(part 1 of 3)
# Autodesk Inventor assembly: printer
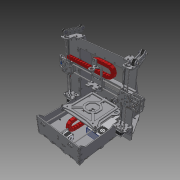
[picture p0: Inventor's stored thumbnail of the model, 180x180]
Saved by Autodesk Inventor 2014 (Build 180170000, 170)
## iProperties
Created: 2013-12-06
Part Number: printer
Document SubType Name: Assembly
Designer: buben
Author: buben
## Documents named in this file (52)
- C:\Users\buben\Documents\GitHub\bacon\inventor files\assemblies\printer.iam
- C:\Users\buben\Documents\GitHub\bacon\inventor files\printer parts\brace_left.ipt
- C:\Users\buben\Documents\GitHub\bacon\inventor files\printer parts\frame.ipt
- C:\Users\buben\Documents\GitHub\bacon\inventor files\printer parts\z_motor_mount.ipt
- C:\Users\buben\Documents\GitHub\bacon\inventor files\printer parts\z_rod_stopper_bottom.ipt
- C:\Users\buben\Documents\GitHub\bacon\inventor files\utils\washer_m4.ipt
- C:\Users\buben\Documents\Inventor\Content Center Files\R2014\en-US\ISO 4762(2)\ISO 4762 - M4 x 20ISO.ipt
- C:\Users\buben\Documents\Inventor\Content Center Files\R2014\en-US\ISO 7040\ISO 7040 - M4.ipt
- C:\Users\buben\Documents\GitHub\bacon\inventor files\3rd party components\nema_17_stepper\Imported Components\NEMA 17\NEMA 17.iam
- C:\Users\buben\Documents\GitHub\bacon\inventor files\utils\washer_m3.ipt
- C:\Users\buben\Documents\Inventor\Content Center Files\R2014\en-US\ISO 4762(2)\ISO 4762 - M3 x 20ISO.ipt
- C:\Users\buben\Documents\GitHub\bacon\inventor files\utils\z_axis_rod.ipt
- C:\Users\buben\Documents\GitHub\bacon\inventor files\printer parts\z_motor_brace.ipt
- C:\Users\buben\Documents\GitHub\bacon\inventor files\utils\z_threaded_rod.ipt
- C:\Users\buben\Documents\GitHub\bacon\inventor files\printer parts\frame_brace_top.ipt
- C:\Users\buben\Documents\GitHub\bacon\inventor files\printer parts\front.ipt
- C:\Users\buben\Documents\GitHub\bacon\inventor files\printer parts\z_axis_top.ipt
- C:\Users\buben\Documents\GitHub\bacon\inventor files\printer parts\bottom.ipt
- C:\Users\buben\Documents\GitHub\bacon\inventor files\printer parts\wiring_brace.ipt
- C:\Users\buben\Documents\GitHub\bacon\inventor files\printer parts\brace_right.ipt
- C:\Users\buben\Documents\GitHub\bacon\inventor files\printer parts\back.ipt
- C:\Users\buben\Documents\GitHub\bacon\inventor files\utils\y_axis_rod.ipt
- C:\Users\buben\Documents\GitHub\bacon\inventor files\utils\z_axis_cable_mount_a.ipt
- C:\Users\buben\Documents\GitHub\bacon\inventor files\assemblies\x_axis.iam
- C:\Users\buben\Documents\GitHub\bacon\inventor files\utils\cable_chain_22.ipt
- C:\Users\buben\Documents\GitHub\bacon\inventor files\utils\z_axis_cable_mount_b.ipt
- C:\Users\buben\Documents\GitHub\bacon\inventor files\assemblies\y_carriage.iam
- C:\Users\buben\Documents\GitHub\bacon\inventor files\utils\y_axis_cable_mount_b.ipt
- C:\Users\buben\Documents\GitHub\bacon\inventor files\utils\x_axis_cable_mount_a.ipt
- C:\Users\buben\Documents\GitHub\bacon\inventor files\3rd party components\switching_power_supply\Imported Components\MW_switching_25A\MW_switching_25A.iam
- C:\Users\buben\Documents\GitHub\bacon\inventor files\3rd party components\bearing_608\Imported Components\608RS\608RS.ipt
- C:\Users\buben\Documents\GitHub\bacon\inventor files\utils\belt_guide.ipt
- C:\Users\buben\Documents\GitHub\bacon\inventor files\utils\washer_m8.ipt
- C:\Users\buben\Documents\GitHub\bacon\inventor files\printer parts\y_carriage_belt_iddler.ipt
- C:\Users\buben\Documents\GitHub\bacon\inventor files\printer parts\y_carriage_belt_iddler_holder.ipt
- C:\Users\buben\Documents\Inventor\Content Center Files\R2014\en-US\ISO 7040\ISO 7040 - M8.ipt
- C:\Users\buben\Documents\Inventor\Content Center Files\R2014\en-US\ISO 4762(2)\ISO 4762 - M8 x 40ISO.ipt
- C:\Users\buben\Documents\Inventor\Content Center Files\R2014\en-US\ISO 4762(2)\ISO 4762 - M4 x 30ISO.ipt
- C:\Users\buben\Documents\GitHub\bacon\inventor files\printer parts\y_motor_mount.ipt
- C:\Users\buben\Documents\GitHub\bacon\inventor files\printer parts\y_motor_mount_brace.ipt
- C:\Users\buben\Documents\GitHub\bacon\inventor files\printer parts\motor_spacer.ipt
- C:\Users\buben\Documents\GitHub\bacon\inventor files\3rd party components\nema_17_stepper\Imported Components\NEMA 17 with T5 Pulley\NEMA 17 with T5 Pulley.iam
- C:\Users\buben\Documents\GitHub\bacon\inventor files\printer parts\rope_mount_a.ipt
- C:\Users\buben\Documents\GitHub\bacon\inventor files\printer parts\rope_mount_b.ipt
- C:\Users\buben\Documents\GitHub\bacon\inventor files\printer parts\z_axis_top_brace.ipt
- C:\Users\buben\Documents\GitHub\bacon\inventor files\printer parts\rope_mount_holder.ipt
- C:\Users\buben\Documents\GitHub\bacon\inventor files\utils\rope_pulley.ipt
- C:\Users\buben\Documents\Inventor\Content Center Files\R2014\en-US\ISO 4762(2)\ISO 4762 - M4 x 35ISO.ipt
- C:\Users\buben\Documents\GitHub\bacon\inventor files\printer parts\z_axis_top_cap.ipt
- C:\Users\buben\Documents\GitHub\bacon\inventor files\printer parts\y_axis_cap.ipt
- C:\Users\buben\Documents\GitHub\bacon\inventor files\3rd party components\iec_plug_socket\Imported Components\IEC inlet\IEC inlet.ipt
- C:\Users\buben\Documents\Inventor\Content Center Files\R2014\en-US\ANSI B18.6.5M(01)\ANSI B18.6.5M - 2.9x1 x 8(4).ipt
## Components (526 placed, 51 different names)
1. brace_left:1 — Mate:1, Mate:2, Flush:1, Mate:3, Mate:4, Mate:5, Mate:71, Mate:73, Flush:6, Flush:7, Mate:80, Flush:8, Mate:85, Mate:111, Mate:113, Mate:115, Mate:177, Mate:179, Mate:181, Mate:241, Mate:243, Mate:245, Mate:247, Mate:249, Mate:276, Mate:277, Mate:278, Mate:279, Mate:280, Mate:281, Mate:282, Mate:283, Mate:284, Mate:285, Mate:367, Mate:395, Mate:396, Mate:398, Mate:400, Mate:427, Mate:665
2. frame:1 — Mate:3, Mate:4, Mate:5, Mate:6, Flush:2, Flush:3, Mate:7, Flush:4, Flush:5, Mate:70, Mate:72, Mate:74, Mate:75, Mate:76, Mate:77, Mate:78, Mate:79, Mate:84, Flush:9, Mate:86, Flush:10, Mate:87, Mate:88, Mate:211, Mate:212, Mate:213, Mate:214, Mate:215, Mate:216, Mate:217, Mate:218, Mate:219, Mate:220, Mate:221, Mate:222, Mate:223, Mate:224, Mate:225, Mate:226, Mate:227, Mate:228, Mate:229, Mate:230, Mate:333, Mate:334, Mate:335, Mate:336, Mate:337, Mate:338, Mate:343, Mate:344, Mate:345, Mate:346, Mate:347, Mate:348, Mate:391, Mate:397, Mate:401, Mate:402, Mate:428, Mate:639, Mate:640, Mate:642, Mate:644, Mate:661, Mate:662, Mate:663, Mate:664, Mate:669, Mate:671, Mate:677, Mate:683
3. z_motor_mount:1 — Mate:6, Flush:2, Flush:3, Mate:8, Mate:9, Mate:10, Mate:14, Mate:15, Mate:16, Mate:17, Mate:44, Mate:45, Mate:46, Mate:47, Mate:52, Mate:53, Mate:54, Mate:55, Insert:13, Mate:63, Mate:64, Mate:65, Mate:339, Mate:340, Mate:341, Mate:342, Mate:359, Mate:361
4. z_motor_mount:2 — Mate:7, Flush:4, Flush:5, Mate:11, Mate:12, Mate:13, Mate:22, Mate:23, Mate:24, Mate:25, Mate:48, Mate:49, Mate:50, Mate:51, Mate:56, Mate:57, Mate:58, Mate:59, Insert:14, Mate:60, Mate:61, Mate:62, Mate:331, Mate:332, Mate:349, Mate:350, Mate:355, Mate:357
5. z_rod_stopper_bottom:1 — Mate:8, Mate:9, Mate:10, Mate:18, Mate:20, Mate:38, Mate:39, Mate:40
6. z_rod_stopper_bottom:2 — Mate:11, Mate:12, Mate:13, Mate:26, Mate:28, Mate:41, Mate:42, Mate:43
7. CSN 02 1702 B B 4,3:1 — Mate:22, Mate:23, Insert:4
8. CSN 02 1702 B B 4,3:2 — Mate:26, Mate:27, Mate:34
9. CSN 02 1702 B B 4,3:3 — Mate:18, Mate:19, Mate:30
10. CSN 02 1702 B B 4,3:4 — Mate:20, Mate:21, Mate:32
11. CSN 02 1702 B B 4,3:5 — Mate:14, Mate:16, Insert:1
12. CSN 02 1702 B B 4,3:6 — Mate:15, Mate:17, Insert:2
13. CSN 02 1702 B B 4,3:7 — Mate:28, Mate:29, Mate:36
14. CSN 02 1702 B B 4,3:8 — Mate:24, Mate:25, Insert:3
15. ISO 4762 M4 x 20:1 — Insert:4, Mate:29, Mate:37
16. ISO 4762 M4 x 20:2 — Insert:3, Mate:27, Mate:35
17. ISO 4762 M4 x 20:3 — Insert:2, Mate:19, Mate:31
18. ISO 4762 M4 x 20:4 — Insert:1, Mate:21, Mate:33
19. DIN EN ISO 7040 M4:1 — Mate:36, Mate:37
20. DIN EN ISO 7040 M4:2 — Mate:34, Mate:35
21. DIN EN ISO 7040 M4:3 — Mate:32, Mate:33
22. DIN EN ISO 7040 M4:4 — Mate:30, Mate:31
23. NEMA 17:1 [sub-assembly] — Mate:38, Mate:39, Mate:40, Mate:66, Mate:67
24. NEMA 17:2 [sub-assembly] — Mate:41, Mate:42, Mate:43, Mate:68, Mate:69
25. CSN 02 1702 B B 3,2:1 — Mate:45, Mate:53, Insert:8
26. CSN 02 1702 B B 3,2:2 — Mate:48, Mate:57, Insert:10
27. CSN 02 1702 B B 3,2:3 — Mate:49, Mate:59, Insert:11
28. CSN 02 1702 B B 3,2:4 — Mate:50, Mate:58, Insert:12
29. CSN 02 1702 B B 3,2:5 — Mate:51, Mate:56, Insert:9
30. CSN 02 1702 B B 3,2:6 — Mate:46, Mate:55, Insert:7
31. CSN 02 1702 B B 3,2:7 — Mate:47, Mate:54, Insert:5
32. CSN 02 1702 B B 3,2:8 — Mate:44, Mate:52, Insert:6
33. ISO 4762 M3 x 20:1 — Insert:12
34. ISO 4762 M3 x 20:2 — Insert:11
35. ISO 4762 M3 x 20:3 — Insert:10
36. ISO 4762 M3 x 20:4 — Insert:9
37. ISO 4762 M3 x 20:5 — Insert:8
38. ISO 4762 M3 x 20:6 — Insert:7
39. ISO 4762 M3 x 20:7 — Insert:6
40. ISO 4762 M3 x 20:8 — Insert:5
41. z_axis_rod:1 — Insert:14, Mate:434
42. z_axis_rod:2 — Insert:13, Mate:433
43. z_motor_brace:1 — Mate:60, Mate:61, Mate:62, Mate:351, Mate:369
44. z_motor_brace:2 — Mate:63, Mate:64, Mate:65, Mate:363, Mate:365
45. z_threaded_rod:1 — Mate:66, Mate:67
46. z_threaded_rod:2 — Mate:68, Mate:69
47. frame_brace_top:1 — Mate:70, Mate:71, Mate:72, Mate:403, Mate:405, Mate:429
48. front:1 — Mate:73, Flush:6, Flush:7, Mate:81, Insert:15, Insert:16, Mate:91, Mate:92, Mate:93, Mate:94, Mate:95, Mate:96, Mate:97, Mate:98, Mate:99, Mate:100, Mate:101, Mate:102, Mate:103, Mate:104, Mate:105, Mate:106, Mate:107, Mate:108, Mate:109, Mate:110, Mate:495, Mate:496, Mate:497, Mate:498, Mate:499, Mate:500, Mate:501, Mate:735, Mate:736, Mate:743, Mate:744, Mate:745, Mate:746, Mate:767, Mate:768, Mate:769, Mate:770
49. z_axis_top:1 — Mate:74, Mate:75, Mate:76, Mate:527, Flush:15, Mate:528, Mate:529, Flush:16, Flush:17, Mate:641, Mate:645, Mate:646, Mate:647, Mate:648, Mate:705, Mate:706, Mate:707, Mate:719, Mate:721
50. z_axis_top:2 — Mate:77, Mate:78, Mate:79, Mate:539, Mate:540, Mate:541, Mate:542, Mate:543, Mate:544, Mate:643, Mate:649, Mate:650, Mate:651, Mate:652, Mate:708, Mate:709, Mate:710, Mate:723, Mate:725
51. bottom:1 — Mate:80, Mate:81, Flush:8, Mate:89, Flush:11, Flush:13, Mate:117, Mate:119, Mate:121, Mate:123, Mate:183, Mate:185, Mate:187, Mate:189, Mate:291, Mate:293, Mate:295, Mate:297, Mate:299, Mate:301, Mate:303, Mate:305, Mate:307, Mate:309, Mate:443, Mate:444, Mate:445
52. wiring_brace:1 — Mate:84, Flush:9, Mate:85, Mate:409, Mate:413
53. wiring_brace:2 — Mate:86, Flush:10, Mate:87, Mate:407, Mate:411
54. brace_right:1 — Mate:88, Mate:89, Flush:11, Mate:90, Flush:12, Mate:125, Mate:127, Mate:129, Mate:171, Mate:173, Mate:175, Mate:231, Mate:233, Mate:235, Mate:237, Mate:239, Mate:271, Mate:272, Mate:273, Mate:274, Mate:275, Mate:286, Mate:287, Mate:288, Mate:289, Mate:290, Mate:353, Mate:392, Mate:393, Mate:394, Mate:399, Mate:446, Mate:675, Mate:795, Mate:796, Mate:797
55. back:1 — Mate:90, Flush:12, Flush:13, Mate:151, Mate:152, Mate:153, Mate:154, Mate:155, Mate:156, Mate:157, Mate:158, Mate:159, Mate:160, Mate:161, Mate:162, Mate:163, Mate:164, Mate:165, Mate:166, Mate:167, Mate:168, Mate:169, Mate:170, Mate:442, Mate:447, Mate:469, Mate:477, Mate:478, Mate:479, Mate:480, Mate:481, Mate:482, Mate:737, Mate:738, Mate:739, Mate:740, Mate:741, Mate:742, Mate:759, Mate:760, Mate:761, Mate:762
56. y_axis_rod:1 — Insert:16, Mate:441
57. y_axis_rod:2 — Insert:15, Mate:440
58. CSN 02 1702 B B 4,3:9 — Mate:97, Mate:107, Insert:23
59. CSN 02 1702 B B 4,3:10 — Mate:98, Mate:108, Insert:24
60. CSN 02 1702 B B 4,3:11 — Mate:99, Mate:109, Insert:25
61. CSN 02 1702 B B 4,3:12 — Mate:129, Mate:130, Mate:149
62. CSN 02 1702 B B 4,3:13 — Mate:94, Mate:104, Insert:20
63. CSN 02 1702 B B 4,3:14 — Mate:95, Mate:105, Insert:21
64. CSN 02 1702 B B 4,3:15 — Mate:96, Mate:106, Insert:22
65. CSN 02 1702 B B 4,3:16 — Mate:93, Mate:103, Insert:19
66. CSN 02 1702 B B 4,3:17 — Mate:92, Mate:102, Insert:18
67. CSN 02 1702 B B 4,3:18 — Mate:91, Mate:101, Insert:17
68. CSN 02 1702 B B 4,3:19 — Mate:127, Mate:128, Mate:147
69. CSN 02 1702 B B 4,3:20 — Mate:117, Mate:118, Mate:137
70. CSN 02 1702 B B 4,3:21 — Mate:115, Mate:116, Mate:135
71. CSN 02 1702 B B 4,3:22 — Mate:100, Mate:110, Insert:26
72. CSN 02 1702 B B 4,3:23 — Mate:125, Mate:126, Mate:145
73. CSN 02 1702 B B 4,3:24 — Mate:121, Mate:122, Mate:141
74. CSN 02 1702 B B 4,3:25 — Mate:113, Mate:114, Mate:133
75. CSN 02 1702 B B 4,3:26 — Mate:123, Mate:124, Mate:143
76. CSN 02 1702 B B 4,3:27 — Mate:119, Mate:120, Mate:139
77. CSN 02 1702 B B 4,3:28 — Mate:111, Mate:112, Mate:131
78. ISO 4762 M4 x 20:5 — Insert:17, Mate:112, Mate:132
79. ISO 4762 M4 x 20:6 — Insert:18, Mate:114, Mate:134
80. ISO 4762 M4 x 20:7 — Insert:19, Mate:116, Mate:136
81. ISO 4762 M4 x 20:8 — Insert:20, Mate:118, Mate:138
82. ISO 4762 M4 x 20:9 — Insert:21, Mate:120, Mate:140
83. ISO 4762 M4 x 20:10 — Insert:22, Mate:122, Mate:142
84. ISO 4762 M4 x 20:11 — Insert:23, Mate:124, Mate:144
85. ISO 4762 M4 x 20:12 — Insert:24, Mate:130, Mate:150
86. ISO 4762 M4 x 20:13 — Insert:25, Mate:128, Mate:148
87. ISO 4762 M4 x 20:14 — Insert:26, Mate:126, Mate:146
88. DIN EN ISO 7040 M4:5 — Mate:131, Mate:132
89. DIN EN ISO 7040 M4:6 — Mate:141, Mate:142
90. DIN EN ISO 7040 M4:7 — Mate:143, Mate:144
91. DIN EN ISO 7040 M4:8 — Mate:147, Mate:148
92. DIN EN ISO 7040 M4:9 — Mate:135, Mate:136
93. DIN EN ISO 7040 M4:10 — Mate:145, Mate:146
94. DIN EN ISO 7040 M4:11 — Mate:149, Mate:150
95. DIN EN ISO 7040 M4:12 — Mate:133, Mate:134
96. DIN EN ISO 7040 M4:13 — Mate:137, Mate:138
97. DIN EN ISO 7040 M4:14 — Mate:139, Mate:140
98. CSN 02 1702 B B 4,3:29 — Mate:151, Mate:168, Insert:29
99. CSN 02 1702 B B 4,3:30 — Mate:152, Mate:169, Insert:28
100. CSN 02 1702 B B 4,3:31 — Mate:160, Mate:161, Insert:36
101. CSN 02 1702 B B 4,3:32 — Mate:153, Mate:170, Insert:27
102. CSN 02 1702 B B 4,3:33 — Mate:154, Mate:167, Insert:30
103. CSN 02 1702 B B 4,3:34 — Mate:159, Mate:162, Insert:35
104. CSN 02 1702 B B 4,3:35 — Mate:155, Mate:166, Insert:31
105. CSN 02 1702 B B 4,3:36 — Mate:156, Mate:165, Insert:32
106. CSN 02 1702 B B 4,3:37 — Mate:157, Mate:164, Insert:33
107. CSN 02 1702 B B 4,3:38 — Mate:158, Mate:163, Insert:34
108. CSN 02 1702 B B 4,3:39 — Mate:171, Mate:172, Mate:205
109. CSN 02 1702 B B 4,3:40 — Mate:175, Mate:176, Mate:209
110. CSN 02 1702 B B 4,3:41 — Mate:173, Mate:174, Mate:207
111. CSN 02 1702 B B 4,3:42 — Mate:177, Mate:178, Mate:191
112. CSN 02 1702 B B 4,3:43 — Mate:181, Mate:182, Mate:195
113. CSN 02 1702 B B 4,3:44 — Mate:187, Mate:188, Mate:201
114. CSN 02 1702 B B 4,3:45 — Mate:179, Mate:180, Mate:193
115. CSN 02 1702 B B 4,3:46 — Mate:183, Mate:184, Mate:197
116. CSN 02 1702 B B 4,3:47 — Mate:185, Mate:186, Mate:199
117. CSN 02 1702 B B 4,3:48 — Mate:189, Mate:190, Mate:203
118. ISO 4762 M4 x 20:15 — Insert:27, Mate:178, Mate:192
119. ISO 4762 M4 x 20:16 — Insert:28, Mate:180, Mate:194
120. ISO 4762 M4 x 20:17 — Insert:29, Mate:182, Mate:196
121. ISO 4762 M4 x 20:18 — Insert:30, Mate:184, Mate:198
122. ISO 4762 M4 x 20:19 — Insert:31, Mate:186, Mate:200
123. ISO 4762 M4 x 20:20 — Insert:32, Mate:188, Mate:202
124. ISO 4762 M4 x 20:21 — Insert:33, Mate:190, Mate:204
125. ISO 4762 M4 x 20:22 — Insert:34, Mate:176, Mate:210
126. ISO 4762 M4 x 20:23 — Insert:35, Mate:174, Mate:208
127. ISO 4762 M4 x 20:24 — Insert:36, Mate:172, Mate:206
128. DIN EN ISO 7040 M4:15 — Mate:193, Mate:194
129. DIN EN ISO 7040 M4:16 — Mate:207, Mate:208
130. DIN EN ISO 7040 M4:17 — Mate:191, Mate:192
131. DIN EN ISO 7040 M4:18 — Mate:201, Mate:202
132. DIN EN ISO 7040 M4:19 — Mate:209, Mate:210
133. DIN EN ISO 7040 M4:20 — Mate:205, Mate:206
134. DIN EN ISO 7040 M4:21 — Mate:203, Mate:204
135. DIN EN ISO 7040 M4:22 — Mate:195, Mate:196
136. DIN EN ISO 7040 M4:23 — Mate:197, Mate:198
137. DIN EN ISO 7040 M4:24 — Mate:199, Mate:200
138. CSN 02 1702 B B 4,3:49 — Mate:211, Mate:226, Insert:37
139. CSN 02 1702 B B 4,3:50 — Mate:213, Mate:228, Insert:39
140. CSN 02 1702 B B 4,3:51 — Mate:214, Mate:229, Insert:40
141. CSN 02 1702 B B 4,3:52 — Mate:215, Mate:230, Insert:41
142. CSN 02 1702 B B 4,3:53 — Mate:216, Mate:221, Insert:42
143. CSN 02 1702 B B 4,3:54 — Mate:217, Mate:222, Insert:43
144. CSN 02 1702 B B 4,3:55 — Mate:218, Mate:223, Insert:44
145. CSN 02 1702 B B 4,3:56 — Mate:219, Mate:224, Insert:45
146. CSN 02 1702 B B 4,3:57 — Mate:220, Mate:225, Insert:46
147. CSN 02 1702 B B 4,3:58 — Mate:247, Mate:248, Mate:267
148. CSN 02 1702 B B 4,3:59 — Mate:212, Mate:227, Insert:38
149. CSN 02 1702 B B 4,3:60 — Mate:231, Mate:232, Mate:251
150. CSN 02 1702 B B 4,3:61 — Mate:233, Mate:234, Mate:253
151. CSN 02 1702 B B 4,3:62 — Mate:235, Mate:236, Mate:255
152. CSN 02 1702 B B 4,3:63 — Mate:237, Mate:238, Mate:257
153. CSN 02 1702 B B 4,3:64 — Mate:239, Mate:240, Mate:259
154. CSN 02 1702 B B 4,3:65 — Mate:241, Mate:242, Mate:261
155. CSN 02 1702 B B 4,3:66 — Mate:243, Mate:244, Mate:263
156. CSN 02 1702 B B 4,3:67 — Mate:245, Mate:246, Mate:265
157. CSN 02 1702 B B 4,3:68 — Mate:249, Mate:250, Mate:269
158. ISO 4762 M4 x 20:25 — Insert:37, Mate:232, Mate:252
159. ISO 4762 M4 x 20:26 — Insert:38, Mate:234, Mate:254
160. ISO 4762 M4 x 20:27 — Insert:39, Mate:236, Mate:256
161. ISO 4762 M4 x 20:28 — Insert:40, Mate:238, Mate:258
162. ISO 4762 M4 x 20:29 — Insert:41, Mate:240, Mate:260
163. ISO 4762 M4 x 20:30 — Insert:42, Mate:242, Mate:262
164. ISO 4762 M4 x 20:31 — Insert:43, Mate:244, Mate:264
165. ISO 4762 M4 x 20:32 — Insert:44, Mate:246, Mate:266
166. ISO 4762 M4 x 20:33 — Insert:45, Mate:248, Mate:268
167. ISO 4762 M4 x 20:34 — Insert:46, Mate:250, Mate:270
168. DIN EN ISO 7040 M4:25 — Mate:251, Mate:252
169. DIN EN ISO 7040 M4:26 — Mate:253, Mate:254
170. DIN EN ISO 7040 M4:27 — Mate:255, Mate:256
171. DIN EN ISO 7040 M4:28 — Mate:261, Mate:262
172. DIN EN ISO 7040 M4:29 — Mate:263, Mate:264
173. DIN EN ISO 7040 M4:30 — Mate:267, Mate:268
174. DIN EN ISO 7040 M4:31 — Mate:269, Mate:270
175. DIN EN ISO 7040 M4:32 — Mate:265, Mate:266
176. DIN EN ISO 7040 M4:33 — Mate:259, Mate:260
177. DIN EN ISO 7040 M4:34 — Mate:257, Mate:258
178. CSN 02 1702 B B 4,3:69 — Mate:271, Mate:290, Insert:51
179. CSN 02 1702 B B 4,3:70 — Mate:272, Mate:289, Insert:50
180. CSN 02 1702 B B 4,3:71 — Mate:273, Mate:288, Insert:49
181. CSN 02 1702 B B 4,3:72 — Mate:274, Mate:287, Insert:48
182. CSN 02 1702 B B 4,3:73 — Mate:275, Mate:286, Insert:47
183. CSN 02 1702 B B 4,3:74 — Mate:276, Mate:281, Insert:56
184. CSN 02 1702 B B 4,3:75 — Mate:277, Mate:282, Insert:55
185. CSN 02 1702 B B 4,3:76 — Mate:278, Mate:283, Insert:54
186. CSN 02 1702 B B 4,3:77 — Mate:279, Mate:284, Insert:53
187. CSN 02 1702 B B 4,3:78 — Mate:280, Mate:285, Insert:52
188. CSN 02 1702 B B 4,3:79 — Mate:303, Mate:304, Mate:317
189. CSN 02 1702 B B 4,3:80 — Mate:305, Mate:306, Mate:315
190. CSN 02 1702 B B 4,3:81 — Mate:307, Mate:308, Mate:313
191. CSN 02 1702 B B 4,3:82 — Mate:309, Mate:310, Mate:311
192. CSN 02 1702 B B 4,3:83 — Mate:301, Mate:302, Mate:319
193. CSN 02 1702 B B 4,3:84 — Mate:299, Mate:300, Mate:329
194. CSN 02 1702 B B 4,3:85 — Mate:297, Mate:298, Mate:325
195. CSN 02 1702 B B 4,3:86 — Mate:295, Mate:296, Mate:327
196. CSN 02 1702 B B 4,3:87 — Mate:293, Mate:294, Mate:323
197. CSN 02 1702 B B 4,3:88 — Mate:291, Mate:292, Mate:321
198. ISO 4762 M4 x 20:35 — Insert:56, Mate:300, Mate:330
199. ISO 4762 M4 x 20:36 — Insert:55, Mate:298, Mate:326
200. ISO 4762 M4 x 20:37 — Insert:54, Mate:296, Mate:328
201. ISO 4762 M4 x 20:38 — Insert:53, Mate:294, Mate:324
202. ISO 4762 M4 x 20:39 — Insert:52, Mate:292, Mate:322
203. ISO 4762 M4 x 20:40 — Insert:51, Mate:302, Mate:320
204. ISO 4762 M4 x 20:41 — Insert:50, Mate:304, Mate:318
205. ISO 4762 M4 x 20:42 — Insert:49, Mate:306, Mate:316
206. ISO 4762 M4 x 20:43 — Insert:48, Mate:308, Mate:314
207. ISO 4762 M4 x 20:44 — Insert:47, Mate:310, Mate:312
208. DIN EN ISO 7040 M4:35 — Mate:329, Mate:330
209. DIN EN ISO 7040 M4:36 — Mate:327, Mate:328
210. DIN EN ISO 7040 M4:37 — Mate:321, Mate:322
211. DIN EN ISO 7040 M4:38 — Mate:317, Mate:318
212. DIN EN ISO 7040 M4:39 — Mate:315, Mate:316
213. DIN EN ISO 7040 M4:40 — Mate:313, Mate:314
214. DIN EN ISO 7040 M4:41 — Mate:311, Mate:312
215. DIN EN ISO 7040 M4:42 — Mate:319, Mate:320
216. DIN EN ISO 7040 M4:43 — Mate:323, Mate:324
217. DIN EN ISO 7040 M4:44 — Mate:325, Mate:326
218. CSN 02 1702 B B 4,3:89 — Mate:340, Mate:341, Insert:65
219. CSN 02 1702 B B 4,3:90 — Mate:339, Mate:342, Insert:66
220. CSN 02 1702 B B 4,3:91 — Mate:338, Mate:345, Insert:64
221. CSN 02 1702 B B 4,3:92 — Mate:337, Mate:344, Insert:63
222. CSN 02 1702 B B 4,3:93 — Mate:336, Mate:343, Insert:62
223. CSN 02 1702 B B 4,3:94 — Mate:335, Mate:348, Insert:61
224. CSN 02 1702 B B 4,3:95 — Mate:334, Mate:347, Insert:59
225. CSN 02 1702 B B 4,3:96 — Mate:333, Mate:346, Insert:60
226. CSN 02 1702 B B 4,3:97 — Mate:332, Mate:349, Insert:57
227. CSN 02 1702 B B 4,3:98 — Mate:331, Mate:350, Insert:58
228. CSN 02 1702 B B 4,3:99 — Mate:367, Mate:368, Mate:385
229. CSN 02 1702 B B 4,3:100 — Mate:369, Mate:370, Mate:375
230. CSN 02 1702 B B 4,3:101 — Mate:365, Mate:366, Mate:383
231. CSN 02 1702 B B 4,3:102 — Mate:363, Mate:364, Mate:381
232. CSN 02 1702 B B 4,3:103 — Mate:361, Mate:362, Mate:389
233. CSN 02 1702 B B 4,3:104 — Mate:359, Mate:360, Mate:387
234. CSN 02 1702 B B 4,3:105 — Mate:357, Mate:358, Mate:373
235. CSN 02 1702 B B 4,3:106 — Mate:355, Mate:356, Mate:371
236. CSN 02 1702 B B 4,3:107 — Mate:353, Mate:354, Mate:379
237. CSN 02 1702 B B 4,3:108 — Mate:351, Mate:352, Mate:377
238. ISO 4762 M4 x 20:45 — Insert:64, Mate:364, Mate:382
239. ISO 4762 M4 x 20:46 — Insert:65, Mate:366, Mate:384
240. ISO 4762 M4 x 20:47 — Insert:66, Mate:368, Mate:386
241. ISO 4762 M4 x 20:48 — Insert:63, Mate:360, Mate:388
242. ISO 4762 M4 x 20:49 — Insert:62, Mate:362, Mate:390
243. ISO 4762 M4 x 20:50 — Insert:61, Mate:370, Mate:376
244. ISO 4762 M4 x 20:51 — Insert:60, Mate:358, Mate:374
245. ISO 4762 M4 x 20:52 — Insert:59, Mate:356, Mate:372
246. ISO 4762 M4 x 20:53 — Insert:58, Mate:354, Mate:380
247. ISO 4762 M4 x 20:54 — Insert:57, Mate:352, Mate:378
248. DIN EN ISO 7040 M4:45 — Mate:389, Mate:390
249. DIN EN ISO 7040 M4:46 — Mate:387, Mate:388
250. DIN EN ISO 7040 M4:47 — Mate:385, Mate:386
251. DIN EN ISO 7040 M4:48 — Mate:383, Mate:384
252. DIN EN ISO 7040 M4:49 — Mate:381, Mate:382
253. DIN EN ISO 7040 M4:50 — Mate:379, Mate:380
254. DIN EN ISO 7040 M4:51 — Mate:377, Mate:378
255. DIN EN ISO 7040 M4:52 — Mate:373, Mate:374
256. DIN EN ISO 7040 M4:53 — Mate:375, Mate:376
257. DIN EN ISO 7040 M4:54 — Mate:371, Mate:372
258. CSN 02 1702 B B 4,3:109 — Mate:393, Mate:394, Insert:67
259. CSN 02 1702 B B 4,3:110 — Mate:397, Mate:402, Insert:69
260. CSN 02 1702 B B 4,3:111 — Mate:398, Mate:400, Insert:71
261. CSN 02 1702 B B 4,3:112 — Mate:407, Mate:408, Mate:415
262. CSN 02 1702 B B 4,3:113 — Mate:403, Mate:404, Mate:425
263. CSN 02 1702 B B 4,3:114 — Mate:395, Mate:396, Insert:72
264. CSN 02 1702 B B 4,3:115 — Mate:392, Mate:399, Insert:70
265. CSN 02 1702 B B 4,3:116 — Mate:405, Mate:406, Mate:419
266. CSN 02 1702 B B 4,3:117 — Mate:411, Mate:412, Mate:417
267. CSN 02 1702 B B 4,3:118 — Mate:413, Mate:414, Mate:421
268. CSN 02 1702 B B 4,3:119 — Mate:409, Mate:410, Mate:423
269. CSN 02 1702 B B 4,3:120 — Mate:391, Mate:401, Insert:68
270. ISO 4762 M4 x 20:55 — Insert:72, Mate:404, Mate:426
271. ISO 4762 M4 x 20:56 — Insert:71, Mate:410, Mate:424
272. ISO 4762 M4 x 20:57 — Insert:70, Mate:408, Mate:416
273. ISO 4762 M4 x 20:58 — Insert:69, Mate:414, Mate:422
274. ISO 4762 M4 x 20:59 — Insert:68, Mate:412, Mate:418
275. ISO 4762 M4 x 20:60 — Insert:67, Mate:406, Mate:420
276. DIN EN ISO 7040 M4:55 — Mate:425, Mate:426
277. DIN EN ISO 7040 M4:56 — Mate:423, Mate:424
278. DIN EN ISO 7040 M4:57 — Mate:421, Mate:422
279. DIN EN ISO 7040 M4:58 — Mate:419, Mate:420
280. DIN EN ISO 7040 M4:59 — Mate:417, Mate:418
281. DIN EN ISO 7040 M4:60 — Mate:415, Mate:416
282. z_axis_cable_mount_a:1 — Mate:427, Mate:428, Mate:429, Insert:96, Angle:24
283. x_axis:1 [sub-assembly] — Mate:433, Mate:434, Mate:435, Flush:14
284. cable_chain_22:1 — Insert:96, Angle:24
285. cable_chain_22:2
286. cable_chain_22:3
287. cable_chain_22:4
288. cable_chain_22:5
289. cable_chain_22:6
290. cable_chain_22:7
291. cable_chain_22:8
292. cable_chain_22:9
293. cable_chain_22:10
294. cable_chain_22:11
295. cable_chain_22:12
296. cable_chain_22:13
297. cable_chain_22:14
298. cable_chain_22:15
299. cable_chain_22:16
300. cable_chain_22:17
301. cable_chain_22:18
302. cable_chain_22:19
303. cable_chain_22:20 — Insert:97, Angle:25
304. z_axis_cable_mount_b:1 — Insert:97, Mate:435, Flush:14, Angle:25
305. y_carriage:1 [sub-assembly] — Mate:436, Mate:437, Mate:438, Mate:440, Mate:441
306. y_axis_cable_mount_b:1 — Mate:436, Mate:437, Mate:438, Insert:121, Angle:65
307. cable_chain_22:22 — Insert:122, Angle:66
308. cable_chain_22:23
309. cable_chain_22:24
310. cable_chain_22:25
311. cable_chain_22:26
312. cable_chain_22:27
313. cable_chain_22:28
314. cable_chain_22:29
315. cable_chain_22:30
316. cable_chain_22:31 — Mate:444
317. cable_chain_22:32
318. cable_chain_22:33
319. cable_chain_22:34
320. cable_chain_22:35
321. cable_chain_22:36
322. cable_chain_22:37
323. cable_chain_22:38
324. cable_chain_22:39
325. cable_chain_22:40
326. cable_chain_22:41
327. cable_chain_22:42
328. cable_chain_22:43
329. cable_chain_22:44 — Insert:121, Angle:65
330. x_axis_cable_mount_a:1 — Insert:122, Angle:66, Mate:442, Mate:443
331. MW_switching_25A:1 [sub-assembly] — Mate:445, Mate:446, Mate:447
332. 608RS:1 — Mate:448, Mate:449, Mate:450, Mate:453, Mate:454, Mate:457, Mate:458
333. belt_guide:1 — Mate:448, Mate:449, Mate:451, Mate:452
334. belt_guide:2 — Mate:450, Mate:451, Mate:452
335. CSN 02 1702 B B 8,4:1 — Mate:453, Mate:454, Mate:455, Mate:456
336. CSN 02 1702 B B 8,4:2 — Mate:455, Mate:456, Mate:461, Mate:462
337. CSN 02 1702 B B 8,4:3 — Mate:457, Mate:458, Mate:459, Mate:460
338. CSN 02 1702 B B 8,4:4 — Mate:459, Mate:460
339. y_carriage_belt_iddler:1 — Mate:461, Mate:462, Mate:463, Mate:464, Mate:465, Mate:472
340. y_carriage_belt_iddler:2 — Mate:466, Mate:467, Mate:468, Mate:469, Mate:470, Mate:471, Mate:477, Mate:478
341. y_carriage_belt_iddler_holder:1 — Mate:463, Mate:464, Mate:465, Mate:466, Mate:467, Mate:468, Mate:483, Mate:484
342. CSN 02 1702 B B 8,4:5 — Mate:470, Mate:471, Insert:123
343. CSN 02 1702 B B 8,4:6 — Mate:472, Mate:474, Mate:475
344. DIN EN ISO 7040 M8:1 — Mate:474, Mate:476
345. ISO 4762 M8 x 40:1 — Insert:123, Mate:475, Mate:476
346. CSN 02 1702 B B 4,3:121 — Mate:483, Mate:485, Mate:487
347. CSN 02 1702 B B 4,3:122 — Mate:484, Mate:486, Mate:489
348. CSN 02 1702 B B 4,3:123 — Mate:480, Mate:481, Insert:125
349. CSN 02 1702 B B 4,3:124 — Mate:479, Mate:482, Insert:124
350. ISO 4762 M4 x 30:1 — Insert:124, Mate:485, Mate:488
351. ISO 4762 M4 x 30:2 — Insert:125, Mate:486, Mate:490
352. DIN EN ISO 7040 M4:61 — Mate:487, Mate:488
353. DIN EN ISO 7040 M4:62 — Mate:489, Mate:490
354. y_motor_mount:1 — Mate:491, Mate:492, Mate:493, Mate:494, Tangent:1, Tangent:2, Mate:495, Mate:496, Mate:502, Mate:503, Mate:508, Mate:519, Mate:520, Mate:521, Mate:522
355. y_motor_mount_brace:1 — Mate:491, Mate:492, Mate:493, Mate:497, Mate:504, Mate:505
356. motor_spacer:1 — Mate:494, Tangent:1, Tangent:2, Mate:516, Mate:517, Mate:518, Mate:523, Mate:524, Mate:525, Mate:526
357. CSN 02 1702 B B 4,3:125 — Mate:504, Mate:507, Mate:512
358. CSN 02 1702 B B 4,3:126 — Mate:508, Mate:509, Mate:514
359. CSN 02 1702 B B 4,3:127 — Mate:498, Mate:501, Insert:127
360. CSN 02 1702 B B 4,3:128 — Mate:499, Mate:500, Insert:126
361. CSN 02 1702 B B 4,3:129 — Mate:505, Mate:506, Mate:510
362. CSN 02 1702 B B 4,3:130 — Mate:502, Mate:503, Insert:128
363. ISO 4762 M4 x 20:61 — Insert:126, Mate:509, Mate:515
364. ISO 4762 M4 x 20:62 — Insert:127, Mate:506, Mate:511
365. ISO 4762 M4 x 20:63 — Insert:128, Mate:507, Mate:513
366. DIN EN ISO 7040 M4:63 — Mate:512, Mate:513
367. DIN EN ISO 7040 M4:64 — Mate:514, Mate:515
368. DIN EN ISO 7040 M4:65 — Mate:510, Mate:511
369. NEMA 17 with T5 Pulley:1 [sub-assembly] — Mate:516, Mate:517, Mate:518
370. CSN 02 1702 B B 3,2:9 — Mate:519, Mate:523, Insert:130
371. CSN 02 1702 B B 3,2:10 — Mate:520, Mate:524, Insert:129
372. CSN 02 1702 B B 3,2:11 — Mate:521, Mate:525, Insert:132
373. CSN 02 1702 B B 3,2:12 — Mate:522, Mate:526, Insert:131
374. ISO 4762 M3 x 20:9 — Insert:132
375. ISO 4762 M3 x 20:10 — Insert:131
376. ISO 4762 M3 x 20:11 — Insert:130
377. ISO 4762 M3 x 20:12 — Insert:129
378. rope_mount_a:1 — Mate:527, Flush:15, Mate:528, Mate:532, Mate:619, Mate:620
379. rope_mount_b:1 — Mate:529, Flush:16, Flush:17, Mate:533, Mate:534, Mate:607, Mate:608, Mate:609, Mate:610, Mate:621, Mate:622, Mate:623, Mate:624
380. rope_mount_holder:1 — Mate:532, Mate:533, Mate:534, Mate:653, Mate:654, Mate:655, Mate:656
381. rope_mount_a:2 — Mate:542, Mate:543, Mate:544, Mate:625, Mate:626
382. rope_mount_b:2 — Mate:539, Mate:540, Mate:541, Mate:545, Mate:546, Mate:547, Mate:611, Mate:612, Mate:613, Mate:614, Mate:615, Mate:616, Mate:617, Mate:618
383. rope_mount_holder:2 — Mate:545, Mate:546, Mate:547, Mate:657, Mate:658, Mate:659, Mate:660
384. 608RS:4 — Mate:550, Mate:556, Mate:559, Mate:564, Mate:565, Mate:566, Mate:567
385. rope_pulley:3 — Mate:557, Mate:558, Mate:559
386. rope_pulley:4 — Mate:550, Mate:556, Mate:557, Mate:558
387. CSN 02 1702 B B 8,4:7 — Mate:560, Mate:561, Mate:564, Mate:565
388. CSN 02 1702 B B 8,4:8 — Mate:560, Mate:561
389. CSN 02 1702 B B 8,4:9 — Mate:562, Mate:563, Mate:566, Mate:567
390. CSN 02 1702 B B 8,4:10 — Mate:562, Mate:563, Mate:613, Mate:614
391. 608RS:5
392. rope_pulley:5
393. rope_pulley:6
394. CSN 02 1702 B B 8,4:11
395. CSN 02 1702 B B 8,4:12
396. CSN 02 1702 B B 8,4:13
397. CSN 02 1702 B B 8,4:14 — Mate:607, Mate:608
398. 608RS:6
399. rope_pulley:7
400. rope_pulley:8
401. CSN 02 1702 B B 8,4:15
402. CSN 02 1702 B B 8,4:16
403. CSN 02 1702 B B 8,4:17
404. CSN 02 1702 B B 8,4:18 — Mate:609, Mate:610
405. 608RS:7
406. rope_pulley:9
407. rope_pulley:10
408. CSN 02 1702 B B 8,4:19
409. CSN 02 1702 B B 8,4:20
410. CSN 02 1702 B B 8,4:21
411. CSN 02 1702 B B 8,4:22 — Mate:611, Mate:612
412. CSN 02 1702 B B 8,4:23 — Mate:626, Mate:628, Mate:631
413. CSN 02 1702 B B 8,4:24 — Mate:625, Mate:627, Mate:633
414. CSN 02 1702 B B 8,4:25 — Mate:623, Mate:624, Insert:136
415. CSN 02 1702 B B 8,4:26 — Mate:621, Mate:622, Insert:135
416. CSN 02 1702 B B 8,4:27 — Mate:620, Mate:630, Mate:635
417. CSN 02 1702 B B 8,4:28 — Mate:619, Mate:629, Mate:637
418. CSN 02 1702 B B 8,4:29 — Mate:617, Mate:618, Insert:134
419. CSN 02 1702 B B 8,4:30 — Mate:615, Mate:616, Insert:133
420. ISO 4762 M8 x 40:2 — Insert:136, Mate:630, Mate:636
421. ISO 4762 M8 x 40:3 — Insert:135, Mate:629, Mate:638
422. ISO 4762 M8 x 40:4 — Insert:134, Mate:628, Mate:632
423. ISO 4762 M8 x 40:5 — Insert:133, Mate:627, Mate:634
424. DIN EN ISO 7040 M8:2 — Mate:637, Mate:638
425. DIN EN ISO 7040 M8:3 — Mate:635, Mate:636
426. DIN EN ISO 7040 M8:4 — Mate:633, Mate:634
427. DIN EN ISO 7040 M8:5 — Mate:631, Mate:632
428. z_axis_top_brace:1 — Mate:642, Mate:643, Mate:644, Mate:673, Mate:681
429. z_axis_top_brace:2 — Mate:639, Mate:640, Mate:641, Mate:667, Mate:679
430. CSN 02 1702 B B 4,3:131 — Mate:651, Mate:652, Insert:139
431. CSN 02 1702 B B 4,3:132 — Mate:659, Mate:660, Insert:146
432. CSN 02 1702 B B 4,3:133 — Mate:657, Mate:658, Insert:145
433. CSN 02 1702 B B 4,3:134 — Mate:655, Mate:656, Insert:143
434. CSN 02 1702 B B 4,3:135 — Mate:645, Mate:646, Insert:137
435. CSN 02 1702 B B 4,3:136 — Mate:649, Mate:650, Insert:140
436. CSN 02 1702 B B 4,3:137 — Mate:647, Mate:648, Insert:138
437. CSN 02 1702 B B 4,3:138 — Mate:653, Mate:654, Insert:144
438. CSN 02 1702 B B 4,3:139 — Mate:661, Mate:662, Insert:141
439. CSN 02 1702 B B 4,3:140 — Mate:671, Mate:672, Mate:701
440. CSN 02 1702 B B 4,3:141 — Mate:675, Mate:676, Mate:703
441. CSN 02 1702 B B 4,3:142 — Mate:665, Mate:666, Mate:685
442. CSN 02 1702 B B 4,3:143 — Mate:673, Mate:674, Mate:697
443. CSN 02 1702 B B 4,3:144 — Mate:669, Mate:670, Mate:687
444. CSN 02 1702 B B 4,3:145 — Mate:667, Mate:668, Mate:691
445. CSN 02 1702 B B 4,3:146 — Mate:663, Mate:664, Insert:142
446. ISO 4762 M4 x 20:64 — Insert:137, Mate:666, Mate:686
447. ISO 4762 M4 x 20:65 — Insert:138, Mate:670, Mate:688
448. ISO 4762 M4 x 20:66 — Insert:139, Mate:672, Mate:702
449. ISO 4762 M4 x 20:67 — Insert:140, Mate:676, Mate:704
450. ISO 4762 M4 x 20:68 — Insert:141, Mate:668, Mate:692
451. ISO 4762 M4 x 20:69 — Insert:142, Mate:674, Mate:698
452. ISO 4762 M4 x 35:1 — Insert:143, Mate:680, Mate:690
453. ISO 4762 M4 x 35:2 — Insert:144, Mate:678, Mate:694
454. ISO 4762 M4 x 35:3 — Insert:145, Mate:682, Mate:700
455. ISO 4762 M4 x 35:4 — Insert:146, Mate:684, Mate:696
456. CSN 02 1702 B B 4,3:147 — Mate:679, Mate:680, Mate:689
457. CSN 02 1702 B B 4,3:148 — Mate:681, Mate:682, Mate:699
458. CSN 02 1702 B B 4,3:149 — Mate:683, Mate:684, Mate:695
459. CSN 02 1702 B B 4,3:150 — Mate:677, Mate:678, Mate:693
460. DIN EN ISO 7040 M4:66 — Mate:691, Mate:692
461. DIN EN ISO 7040 M4:67 — Mate:693, Mate:694
462. DIN EN ISO 7040 M4:68 — Mate:695, Mate:696
463. DIN EN ISO 7040 M4:69 — Mate:697, Mate:698
464. DIN EN ISO 7040 M4:70 — Mate:701, Mate:702
465. DIN EN ISO 7040 M4:71 — Mate:685, Mate:686
466. DIN EN ISO 7040 M4:72 — Mate:687, Mate:688
467. DIN EN ISO 7040 M4:73 — Mate:689, Mate:690
468. DIN EN ISO 7040 M4:74 — Mate:699, Mate:700
469. DIN EN ISO 7040 M4:75 — Mate:703, Mate:704
470. z_axis_top_cap:1 — Mate:705, Mate:706, Mate:707, Mate:711, Mate:712, Mate:713, Mate:714
471. z_axis_top_cap:2 — Mate:708, Mate:709, Mate:710, Mate:715, Mate:716, Mate:717, Mate:718
472. CSN 02 1702 B B 4,3:151 — Mate:715, Mate:716, Insert:149
473. CSN 02 1702 B B 4,3:152 — Mate:717, Mate:718, Insert:150
474. CSN 02 1702 B B 4,3:153 — Mate:712, Mate:713, Insert:148
475. CSN 02 1702 B B 4,3:154 — Mate:711, Mate:714, Insert:147
476. ISO 4762 M4 x 20:70 — Insert:150, Mate:724, Mate:732
477. ISO 4762 M4 x 20:71 — Insert:149, Mate:726, Mate:734
478. ISO 4762 M4 x 20:72 — Insert:148, Mate:720, Mate:730
479. ISO 4762 M4 x 20:73 — Insert:147, Mate:722, Mate:728
480. CSN 02 1702 B B 4,3:155 — Mate:719, Mate:720, Mate:729
481. CSN 02 1702 B B 4,3:156 — Mate:721, Mate:722, Mate:727
482. CSN 02 1702 B B 4,3:157 — Mate:723, Mate:724, Mate:731
483. CSN 02 1702 B B 4,3:158 — Mate:725, Mate:726, Mate:733
484. DIN EN ISO 7040 M4:76 — Mate:727, Mate:728
485. DIN EN ISO 7040 M4:77 — Mate:729, Mate:730
486. DIN EN ISO 7040 M4:78 — Mate:731, Mate:732
487. DIN EN ISO 7040 M4:79 — Mate:733, Mate:734
488. y_axis_cap:1 — Mate:735, Mate:745, Mate:746, Mate:747, Mate:748, Mate:763, Mate:764
489. y_axis_cap:2 — Mate:736, Mate:743, Mate:744, Mate:749, Mate:750, Mate:765, Mate:766
490. y_axis_cap:3 — Mate:737, Mate:741, Mate:742, Mate:751, Mate:752, Mate:753, Mate:754
491. y_axis_cap:4 — Mate:738, Mate:739, Mate:740, Mate:755, Mate:756, Mate:757, Mate:758
492. CSN 02 1702 B B 4,3:159 — Mate:750, Mate:766, Insert:154
493. CSN 02 1702 B B 4,3:160 — Mate:749, Mate:765, Insert:153
494. CSN 02 1702 B B 4,3:161 — Mate:748, Mate:764, Insert:152
495. CSN 02 1702 B B 4,3:162 — Mate:747, Mate:763, Insert:151
496. CSN 02 1702 B B 4,3:163 — Mate:751, Mate:752, Insert:155
497. CSN 02 1702 B B 4,3:164 — Mate:753, Mate:754, Insert:156
498. CSN 02 1702 B B 4,3:165 — Mate:755, Mate:756, Insert:158
499. CSN 02 1702 B B 4,3:166 — Mate:757, Mate:758, Insert:157
500. CSN 02 1702 B B 4,3:167 — Mate:759, Mate:777, Mate:793
501. CSN 02 1702 B B 4,3:168 — Mate:760, Mate:778, Mate:791
502. CSN 02 1702 B B 4,3:169 — Mate:761, Mate:776, Mate:789
503. CSN 02 1702 B B 4,3:170 — Mate:762, Mate:775, Mate:787
504. CSN 02 1702 B B 4,3:171 — Mate:767, Mate:771, Mate:779
505. CSN 02 1702 B B 4,3:172 — Mate:768, Mate:772, Mate:781
506. CSN 02 1702 B B 4,3:173 — Mate:769, Mate:774, Mate:783
507. CSN 02 1702 B B 4,3:174 — Mate:770, Mate:773, Mate:785
508. ISO 4762 M4 x 20:74 — Insert:151, Mate:773, Mate:786
509. ISO 4762 M4 x 20:75 — Insert:152, Mate:774, Mate:784
510. ISO 4762 M4 x 20:76 — Insert:153, Mate:772, Mate:782
511. ISO 4762 M4 x 20:77 — Insert:154, Mate:771, Mate:780
512. ISO 4762 M4 x 20:78 — Insert:155, Mate:775, Mate:788
513. ISO 4762 M4 x 20:79 — Insert:156, Mate:776, Mate:790
514. ISO 4762 M4 x 20:80 — Insert:157, Mate:778, Mate:792
515. ISO 4762 M4 x 20:81 — Insert:158, Mate:777, Mate:794
516. DIN EN ISO 7040 M4:80 — Mate:785, Mate:786
517. DIN EN ISO 7040 M4:81 — Mate:783, Mate:784
518. DIN EN ISO 7040 M4:82 — Mate:781, Mate:782
519. DIN EN ISO 7040 M4:83 — Mate:779, Mate:780
520. DIN EN ISO 7040 M4:84 — Mate:787, Mate:788
521. DIN EN ISO 7040 M4:85 — Mate:793, Mate:794
522. DIN EN ISO 7040 M4:86 — Mate:791, Mate:792
523. DIN EN ISO 7040 M4:87 — Mate:789, Mate:790
524. IEC inlet:1 — Mate:795, Mate:796, Mate:797, Insert:159, Insert:160
525. Cross Recessed Flat Countersunk Head Tapping Screw - Type AB - Type IA - Metric 2,9 x 1 x 8:1 — Insert:159
526. Cross Recessed Flat Countersunk Head Tapping Screw - Type AB - Type IA - Metric 2,9 x 1 x 8:2 — Insert:160
## Relationships (996: Mate 777, Insert 155, Angle 45, Flush 17, Tangent 2)
- Mate:1: brace_left:1
- Mate:2: brace_left:1
- Flush:1: brace_left:1
- Mate:3: brace_left:1 ↔ frame:1
- Mate:4: brace_left:1 ↔ frame:1
- Mate:5: brace_left:1 ↔ frame:1
- Mate:6: frame:1 ↔ z_motor_mount:1
- Flush:2: frame:1 ↔ z_motor_mount:1
- Flush:3: frame:1 ↔ z_motor_mount:1
- Mate:7: frame:1 ↔ z_motor_mount:2
- Flush:4: frame:1 ↔ z_motor_mount:2
- Flush:5: frame:1 ↔ z_motor_mount:2
- Mate:8: z_motor_mount:1 ↔ z_rod_stopper_bottom:1
- Mate:9: z_motor_mount:1 ↔ z_rod_stopper_bottom:1
- Mate:10: z_motor_mount:1 ↔ z_rod_stopper_bottom:1
- Mate:11: z_motor_mount:2 ↔ z_rod_stopper_bottom:2
- Mate:12: z_motor_mount:2 ↔ z_rod_stopper_bottom:2
- Mate:13: z_motor_mount:2 ↔ z_rod_stopper_bottom:2
- Mate:14: z_motor_mount:1 ↔ CSN 02 1702 B B 4,3:5
- Mate:15: z_motor_mount:1 ↔ CSN 02 1702 B B 4,3:6
- Mate:16: z_motor_mount:1 ↔ CSN 02 1702 B B 4,3:5